# Autodesk Inventor assembly: TurretAssembly
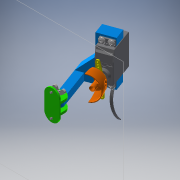
[picture p0: Inventor's stored thumbnail of the model, 180x180]
Saved by Autodesk Inventor 2016 (Build 200138000, 138)
## iProperties
Created: 2016-04-17
Part Number: TurretAssembly
Document SubType Name: Assembly
Designer: amenoni
Author: amenoni
## Documents named in this file (10)
- Z:\Desarrollo\WetMaths\wetMaths-Arduino\wetMaths\HwDesigns\TurretAssembly.iam
- Z:\Desarrollo\WetMaths\wetMaths-Arduino\wetMaths\HwDesigns\turretSupport.ipt
- Z:\Desarrollo\WetMaths\wetMaths-Arduino\wetMaths\HwDesigns\TurretServoSupport.ipt
- Z:\Desarrollo\WetMaths\wetMaths-Arduino\wetMaths\HwDesigns\Futaba S3004.ipt
- Z:\Desarrollo\WetMaths\wetMaths-Arduino\wetMaths\HwDesigns\CanNozzle.ipt
- Z:\Desarrollo\WetMaths\wetMaths-Arduino\wetMaths\HwDesigns\Servo_arm_np1.ipt
- \\psf\Home\Documents\Inventor\Content Center Files\R2016\en-US\AS 1427(05)\AS 1427 - M2.5 x 20(5) II.ipt
- \\psf\Home\Documents\Inventor\Content Center Files\R2016\en-US\KS B 1014\KS B 1014 - M 2.5.ipt
- \\psf\Home\Documents\Inventor\Content Center Files\R2016\en-US\AS 1427(05)\AS 1427 - M2.5 x 4(5) II.ipt
- \\psf\Home\Documents\Inventor\Content Center Files\R2016\en-US\AS 1427(05)\AS 1427 - M4 x 6(5) II.ipt
## Components (13 placed, 9 different names)
1. turretSupport:1 — Mate:1, Mate:2, Mate:11, Mate:12, Mate:14, Insert:1, Insert:2
2. TurretServoSupport:1 — Mate:1, Mate:2, Mate:3, Mate:4, Mate:5
3. Futaba S3004:1 — Mate:3, Mate:4, Mate:5, Mate:6, Mate:7, Insert:3, Mate:15, Mate:16, Insert:4, Insert:5
4. CanNozzle:1 — Mate:8, Mate:9, Mate:10
5. Servo_arm_np1:1 — Mate:6, Mate:7, Mate:8, Mate:9, Mate:10
6. AS 1427 H - Metric M2.5 x 20:1 — Mate:11, Mate:12, Mate:13
7. KS B 1014 - Metric M 2.5:1 — Mate:13, Mate:14
8. AS 1427 H - Metric M2.5 x 4:1 — Insert:1
9. AS 1427 H - Metric M2.5 x 4:2 — Insert:2
10. AS 1427 H - Metric M4 x 6:1 — Insert:3
11. AS 1427 H - Metric M4 x 6:2 — Mate:15, Mate:16
12. AS 1427 H - Metric M4 x 6:3 — Insert:4
13. AS 1427 H - Metric M4 x 6:4 — Insert:5
## Relationships (21: Mate 16, Insert 5)
- Mate:1: turretSupport:1 ↔ TurretServoSupport:1
- Mate:2: turretSupport:1 ↔ TurretServoSupport:1
- Mate:3: TurretServoSupport:1 ↔ Futaba S3004:1
- Mate:4: TurretServoSupport:1 ↔ Futaba S3004:1
- Mate:5: TurretServoSupport:1 ↔ Futaba S3004:1
- Mate:6: Futaba S3004:1 ↔ Servo_arm_np1:1
- Mate:7: Futaba S3004:1 ↔ Servo_arm_np1:1
- Mate:8: CanNozzle:1 ↔ Servo_arm_np1:1
- Mate:9: CanNozzle:1 ↔ Servo_arm_np1:1
- Mate:10: CanNozzle:1 ↔ Servo_arm_np1:1
- Mate:11: turretSupport:1 ↔ AS 1427 H - Metric M2.5 x 20:1
- Mate:12: turretSupport:1 ↔ AS 1427 H - Metric M2.5 x 20:1
- Mate:13: AS 1427 H - Metric M2.5 x 20:1 ↔ KS B 1014 - Metric M 2.5:1
- Mate:14: turretSupport:1 ↔ KS B 1014 - Metric M 2.5:1
- Insert:1: turretSupport:1 ↔ AS 1427 H - Metric M2.5 x 4:1
- Insert:2: turretSupport:1 ↔ AS 1427 H - Metric M2.5 x 4:2
- Insert:3: Futaba S3004:1 ↔ AS 1427 H - Metric M4 x 6:1
- Mate:15: Futaba S3004:1 ↔ AS 1427 H - Metric M4 x 6:2
- Mate:16: Futaba S3004:1 ↔ AS 1427 H - Metric M4 x 6:2
- Insert:4: Futaba S3004:1 ↔ AS 1427 H - Metric M4 x 6:3
- Insert:5: Futaba S3004:1 ↔ AS 1427 H - Metric M4 x 6:4
